# Autodesk Inventor assembly: final Assembly
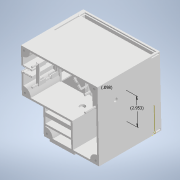
[picture p0: Inventor's stored thumbnail of the model, 180x180]
Saved by Autodesk Inventor 2022 (Build 260153000, 153)
## iProperties
Created: 2022-10-21
Part Number: final Assembly
Document SubType Name: Assembly
Designer: yashm
Author: yashm
## Documents named in this file (6)
- C:\Yash\Raman 2.O\final Assembly.iam
- C:\Yash\Raman 2.O\Box.ipt
- C:\Yash\Raman 2.O\Stand Lower covet.ipt
- C:\Yash\Raman 2.O\Stand Upper covet.ipt
- C:\Yash\Raman 2.O\standlower.ipt
- C:\Yash\Raman 2.O\standupper.ipt
## Components (5 placed, 5 different names)
1. Box:1 — Angle:1, Insert:1, Insert:2, Angle:2
2. Stand Lower covet:1 — Mate:1, Mate:2, Angle:1, Insert:1
3. Stand Upper covet:1 — Mate:1, Mate:2
4. standlower:1 — Mate:3, Mate:4, Insert:2, Angle:2
5. standupper:1 — Mate:3, Mate:4
## Relationships (8: Mate 4, Angle 2, Insert 2)
- Mate:1: Stand Lower covet:1 ↔ Stand Upper covet:1
- Mate:2: Stand Lower covet:1 ↔ Stand Upper covet:1
- Angle:1 (0 deg): Box:1 ↔ Stand Lower covet:1
- Insert:1: Box:1 ↔ Stand Lower covet:1
- Mate:3: standlower:1 ↔ standupper:1
- Mate:4: standlower:1 ↔ standupper:1
- Insert:2: Box:1 ↔ standlower:1
- Angle:2 (0 deg): Box:1 ↔ standlower:1
